# Autodesk Inventor assembly: Top Conveyor Roller Wheel Assembly
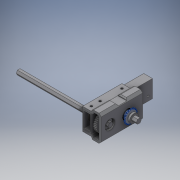
[picture p0: Inventor's stored thumbnail of the model, 180x180]
Saved by Autodesk Inventor 2018 (Build 220112000, 112)
## iProperties
Created: 2020-02-21
Part Number: Top Conveyor Roller Wheel Assembly
Document SubType Name: Assembly
Designer: T3500STATIC
Author: T3500STATIC
## Documents named in this file (11)
- C:\Users\T3500STATIC\Documents\GitHub\2020CAD\Gabriel Inventor Files (Shooter, Drivebase)\Shooter Curve Assembly\Part Files\Top Conveyor Roller Wheel Assembly.iam
- C:\Users\T3500STATIC\Documents\GitHub\2020CAD\Gabriel Inventor Files (Shooter, Drivebase)\Shooter Curve Assembly\Part Files\Top Roller Wheel Mount.ipt
- C:\Users\T3500STATIC\Documents\GitHub\2020CAD\Gabriel Inventor Files (Shooter, Drivebase)\Shooter Curve Assembly\Part Files\_18t_Aluminum_Hub_Sprocket_25_Chain_1_2_Hex_Bore_217-3488.ipt
- C:\Users\T3500STATIC\Documents\GitHub\2020CAD\Gabriel Inventor Files (Shooter, Drivebase)\Drivebase Assembly\Part Files\FR8ZZ Hex Bearing.ipt
- C:\Users\T3500STATIC\Documents\GitHub\2020CAD\Gabriel Inventor Files (Shooter, Drivebase)\Shooter Curve Assembly\Part Files\40t_Aluminum_Spur_Gear_20_DP_1_2_Hex_Bore_217-2708.ipt
- C:\Users\T3500STATIC\Documents\GitHub\2020CAD\Gabriel Inventor Files (Shooter, Drivebase)\Shooter Curve Assembly\Part Files\1_8_Acetal_Spacer_-_1_2_Hex_217-2758.ipt
- C:\Users\T3500STATIC\Documents\GitHub\2020CAD\Gabriel Inventor Files (Shooter, Drivebase)\Shooter Curve Assembly\Part Files\1_2_Acetal_Spacer_-_1_2_Hex_217-3261.ipt
- C:\Users\T3500STATIC\Documents\GitHub\2020CAD\Gabriel Inventor Files (Shooter, Drivebase)\Shooter Curve Assembly\Part Files\Clamping_Shaft_Collar_-_1_2_Hex_ID_217-2737.ipt
- C:\Users\T3500STATIC\Documents\GitHub\2020CAD\Gabriel Inventor Files (Shooter, Drivebase)\Shooter Curve Assembly\Part Files\10.5 in Hex Shaft Top Roller Wheel.ipt
- C:\Users\T3500STATIC\Documents\GitHub\2020CAD\Gabriel Inventor Files (Shooter, Drivebase)\Shooter Curve Assembly\Part Files\4in Hex Shaft Top Roller Wheel.ipt
- C:\Users\T3500STATIC\Documents\GitHub\2020CAD\Gabriel Inventor Files (Shooter, Drivebase)\Shooter Curve Assembly\Part Files\Gearbox Cover.ipt
## Components (19 placed, 10 different names)
1. Top Roller Wheel Mount:1 — Mate:1, Mate:2, Mate:3, Mate:4, Mate:8, Mate:9, Mate:10, Mate:11, Mate:35, Mate:36, Flush:21, Flush:22
2. _18t_Aluminum_Hub_Sprocket_25_Chain_1_2_Hex_Bore_217-3488:1 — Mate:19, Flush:15, Flush:16, Flush:17, Flush:18, Mate:20
3. FR8ZZ Hex Bearing:1 — Mate:2, Mate:9, Flush:1, Flush:2, Flush:5, Flush:6, Mate:12, Mate:22, Mate:23
4. FR8ZZ Hex Bearing:2 — Mate:1, Mate:8, Flush:3, Flush:4, Flush:7, Flush:8, Mate:14, Mate:24, Mate:25
5. FR8ZZ Hex Bearing:3 — Mate:4, Mate:11
6. FR8ZZ Hex Bearing:4 — Mate:3, Mate:10, Flush:20, Mate:28
7. 40t_Aluminum_Spur_Gear_20_DP_1_2_Hex_Bore_217-2708:1 — Flush:1, Flush:2, Mate:13, Flush:9, Flush:10, Mate:21
8. 40t_Aluminum_Spur_Gear_20_DP_1_2_Hex_Bore_217-2708:2 — Flush:3, Flush:4, Mate:15, Flush:13, Flush:14, Mate:18, Flush:15, Flush:16
9. 1_8_Acetal_Spacer_-_1_2_Hex_217-2758:1 — Flush:7, Flush:8, Mate:14, Mate:15
10. 1_8_Acetal_Spacer_-_1_2_Hex_217-2758:2 — Flush:5, Flush:6, Mate:12, Mate:13
11. 1_8_Acetal_Spacer_-_1_2_Hex_217-2758:3 — Mate:26, Mate:27, Mate:28, Mate:31
12. 1_8_Acetal_Spacer_-_1_2_Hex_217-2758:6 — Flush:17, Flush:18, Mate:20, Mate:34
13. 1_2_Acetal_Spacer_-_1_2_Hex_217-3261:1 — Flush:13, Flush:14, Mate:18, Mate:19
14. Clamping_Shaft_Collar_-_1_2_Hex_ID_217-2737:1 — Flush:9, Flush:10, Mate:21, Flush:19
15. 10.5 in Hex Shaft Top Roller Wheel:1 — Mate:22, Mate:23, Flush:19
16. 4in Hex Shaft Top Roller Wheel:1 — Mate:24, Mate:25, Flush:20, Mate:26, Mate:27, Mate:29, Mate:30, Mate:32, Mate:33
17. Clamping_Shaft_Collar_-_1_2_Hex_ID_217-2737:2 — Mate:29, Mate:30, Mate:31
18. Clamping_Shaft_Collar_-_1_2_Hex_ID_217-2737:3 — Mate:32, Mate:33, Mate:34
19. Gearbox Cover:1 — Mate:35, Mate:36, Flush:21, Flush:22
## Relationships (51: Mate 31, Flush 20)
- Mate:1: Top Roller Wheel Mount:1 ↔ FR8ZZ Hex Bearing:2
- Mate:2: Top Roller Wheel Mount:1 ↔ FR8ZZ Hex Bearing:1
- Mate:3: Top Roller Wheel Mount:1 ↔ FR8ZZ Hex Bearing:4
- Mate:4: Top Roller Wheel Mount:1 ↔ FR8ZZ Hex Bearing:3
- Mate:8: Top Roller Wheel Mount:1 ↔ FR8ZZ Hex Bearing:2
- Mate:9: Top Roller Wheel Mount:1 ↔ FR8ZZ Hex Bearing:1
- Mate:10: Top Roller Wheel Mount:1 ↔ FR8ZZ Hex Bearing:4
- Mate:11: Top Roller Wheel Mount:1 ↔ FR8ZZ Hex Bearing:3
- Flush:1: FR8ZZ Hex Bearing:1 ↔ 40t_Aluminum_Spur_Gear_20_DP_1_2_Hex_Bore_217-2708:1
- Flush:2: FR8ZZ Hex Bearing:1 ↔ 40t_Aluminum_Spur_Gear_20_DP_1_2_Hex_Bore_217-2708:1
- Flush:3: FR8ZZ Hex Bearing:2 ↔ 40t_Aluminum_Spur_Gear_20_DP_1_2_Hex_Bore_217-2708:2
- Flush:4: FR8ZZ Hex Bearing:2 ↔ 40t_Aluminum_Spur_Gear_20_DP_1_2_Hex_Bore_217-2708:2
- Flush:5: FR8ZZ Hex Bearing:1 ↔ 1_8_Acetal_Spacer_-_1_2_Hex_217-2758:2
- Flush:6: FR8ZZ Hex Bearing:1 ↔ 1_8_Acetal_Spacer_-_1_2_Hex_217-2758:2
- Mate:12: FR8ZZ Hex Bearing:1 ↔ 1_8_Acetal_Spacer_-_1_2_Hex_217-2758:2
- Mate:13: 40t_Aluminum_Spur_Gear_20_DP_1_2_Hex_Bore_217-2708:1 ↔ 1_8_Acetal_Spacer_-_1_2_Hex_217-2758:2
- Flush:7: FR8ZZ Hex Bearing:2 ↔ 1_8_Acetal_Spacer_-_1_2_Hex_217-2758:1
- Flush:8: FR8ZZ Hex Bearing:2 ↔ 1_8_Acetal_Spacer_-_1_2_Hex_217-2758:1
- Mate:14: FR8ZZ Hex Bearing:2 ↔ 1_8_Acetal_Spacer_-_1_2_Hex_217-2758:1
- Mate:15: 40t_Aluminum_Spur_Gear_20_DP_1_2_Hex_Bore_217-2708:2 ↔ 1_8_Acetal_Spacer_-_1_2_Hex_217-2758:1
- Flush:9: 40t_Aluminum_Spur_Gear_20_DP_1_2_Hex_Bore_217-2708:1 ↔ Clamping_Shaft_Collar_-_1_2_Hex_ID_217-2737:1
- Flush:10: 40t_Aluminum_Spur_Gear_20_DP_1_2_Hex_Bore_217-2708:1 ↔ Clamping_Shaft_Collar_-_1_2_Hex_ID_217-2737:1
- Flush:13: 40t_Aluminum_Spur_Gear_20_DP_1_2_Hex_Bore_217-2708:2 ↔ 1_2_Acetal_Spacer_-_1_2_Hex_217-3261:1
- Flush:14: 40t_Aluminum_Spur_Gear_20_DP_1_2_Hex_Bore_217-2708:2 ↔ 1_2_Acetal_Spacer_-_1_2_Hex_217-3261:1
- Mate:18: 40t_Aluminum_Spur_Gear_20_DP_1_2_Hex_Bore_217-2708:2 ↔ 1_2_Acetal_Spacer_-_1_2_Hex_217-3261:1
- Mate:19: _18t_Aluminum_Hub_Sprocket_25_Chain_1_2_Hex_Bore_217-3488:1 ↔ 1_2_Acetal_Spacer_-_1_2_Hex_217-3261:1
- Flush:15: _18t_Aluminum_Hub_Sprocket_25_Chain_1_2_Hex_Bore_217-3488:1 ↔ 40t_Aluminum_Spur_Gear_20_DP_1_2_Hex_Bore_217-2708:2
- Flush:16: _18t_Aluminum_Hub_Sprocket_25_Chain_1_2_Hex_Bore_217-3488:1 ↔ 40t_Aluminum_Spur_Gear_20_DP_1_2_Hex_Bore_217-2708:2
- Flush:17: _18t_Aluminum_Hub_Sprocket_25_Chain_1_2_Hex_Bore_217-3488:1 ↔ 1_8_Acetal_Spacer_-_1_2_Hex_217-2758:6
- Flush:18: _18t_Aluminum_Hub_Sprocket_25_Chain_1_2_Hex_Bore_217-3488:1 ↔ 1_8_Acetal_Spacer_-_1_2_Hex_217-2758:6
- Mate:20: _18t_Aluminum_Hub_Sprocket_25_Chain_1_2_Hex_Bore_217-3488:1 ↔ 1_8_Acetal_Spacer_-_1_2_Hex_217-2758:6
- Mate:21: 40t_Aluminum_Spur_Gear_20_DP_1_2_Hex_Bore_217-2708:1 ↔ Clamping_Shaft_Collar_-_1_2_Hex_ID_217-2737:1
- Mate:22: FR8ZZ Hex Bearing:1 ↔ 10.5 in Hex Shaft Top Roller Wheel:1
- Mate:23: FR8ZZ Hex Bearing:1 ↔ 10.5 in Hex Shaft Top Roller Wheel:1
- Flush:19 (-6.35 mm): Clamping_Shaft_Collar_-_1_2_Hex_ID_217-2737:1 ↔ 10.5 in Hex Shaft Top Roller Wheel:1
- Mate:24: FR8ZZ Hex Bearing:2 ↔ 4in Hex Shaft Top Roller Wheel:1
- Mate:25: FR8ZZ Hex Bearing:2 ↔ 4in Hex Shaft Top Roller Wheel:1
- Flush:20 (-12.7 mm): FR8ZZ Hex Bearing:4 ↔ 4in Hex Shaft Top Roller Wheel:1
- Mate:26: 1_8_Acetal_Spacer_-_1_2_Hex_217-2758:3 ↔ 4in Hex Shaft Top Roller Wheel:1
- Mate:27: 1_8_Acetal_Spacer_-_1_2_Hex_217-2758:3 ↔ 4in Hex Shaft Top Roller Wheel:1
- Mate:28: FR8ZZ Hex Bearing:4 ↔ 1_8_Acetal_Spacer_-_1_2_Hex_217-2758:3
- Mate:29: 4in Hex Shaft Top Roller Wheel:1 ↔ Clamping_Shaft_Collar_-_1_2_Hex_ID_217-2737:2
- Mate:30: 4in Hex Shaft Top Roller Wheel:1 ↔ Clamping_Shaft_Collar_-_1_2_Hex_ID_217-2737:2
- Mate:31: 1_8_Acetal_Spacer_-_1_2_Hex_217-2758:3 ↔ Clamping_Shaft_Collar_-_1_2_Hex_ID_217-2737:2
- Mate:32: 4in Hex Shaft Top Roller Wheel:1 ↔ Clamping_Shaft_Collar_-_1_2_Hex_ID_217-2737:3
- Mate:33: 4in Hex Shaft Top Roller Wheel:1 ↔ Clamping_Shaft_Collar_-_1_2_Hex_ID_217-2737:3
- Mate:34: 1_8_Acetal_Spacer_-_1_2_Hex_217-2758:6 ↔ Clamping_Shaft_Collar_-_1_2_Hex_ID_217-2737:3
- Mate:35: Top Roller Wheel Mount:1 ↔ Gearbox Cover:1
- Mate:36: Top Roller Wheel Mount:1 ↔ Gearbox Cover:1
- Flush:21: Top Roller Wheel Mount:1 ↔ Gearbox Cover:1
- Flush:22: Top Roller Wheel Mount:1 ↔ Gearbox Cover:1
